# Autodesk Inventor assembly: FY 503 M
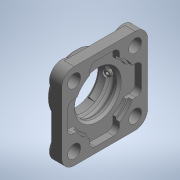
[picture p0: Inventor's stored thumbnail of the model, 180x180]
Saved by Autodesk Inventor 2020 (Build 240168000, 168)
## iProperties
Part Number: FY 503 M
Catalog Web Link: www.cadenas.de
Description: AFC_001-002_AFV_001-Square flanged housings for Y-bearings
Vendor: SKF
Document SubType Name: Assembly
Designer: partserver
Manufacturer: SKF
Mass: 280 g
Surface Area: 199.425 cm^2
Volume: 41.7862 cm^3
Density: 6.70078 g/cm^3
Category: PARTsolutions
Company: SKF
PSOL_IDENT_0: {$CADENAS_DATA\23d-libs\skf\bearings_units_and_housings\bearing_units\ball_bearing_units\y-housings\
PSOL_IDENT_1: afc_001-002_afv_001.prj},190 {VTYP=3D},{STYP=ASSTAB},{NB=FY 503 M},{LINA=FY 503 M},{NN=AFC_001-002_A
PSOL_IDENT_2: FV_001},{DATE=20.08.2020 13:45:12},{GEOMDATE=21.06.2019 12:06:37},{VERSION=},{LINEID=9370},{WBVAR=CO
PSOL_IDENT_3: VER},{WBNUMERIC=}  {NB=FY 503 M},{LINA=FY 503 M},{KT=DUMMY},{PRODUCTID=212600503},{DESIGNATION=FY 50
PSOL_IDENT_4: 3 M},{COVER=},{D=40.000},{DA=55.600},{DB1=50.000},{DB2=53.000},{DB=MIN},{A=26.000},{A1=11.000},{A2=1
PSOL_IDENT_5: 7.000},{A3=3.200},{A5=MIN},{J=54.000},{L=76.000},{N=11.500},{RG=1/4-28 UNF},{R1=19.000},{DN=6.500},{
PSOL_IDENT_6: SWN=7.000},{GN=1/4-28 SAE-LT},{J6=66.000},{J7=14.500},{N4=4.000},{MASS=0.280},{G=10.000},{GIN=0.375}
PSOL_IDENT_7: ,{HOUSING=},{EC=},{AEC=MIN},{DEC=MIN},{D1EC=MIN},{D2EC=MIN},{PPATH=square_flanged_housings_parts/afc
PSOL_IDENT_8: _001-002_afv_001_asmtpl.prj},{DESIGN=fy},{ECALG= '', 'No end cover'},{E=12},{TC=FY 503 M}
NB: FY 503 M
NN: AFC_001-002_AFV_001
NT: Square flanged housings for Y-bearings
NBSYN: $TC.
LINA: FY 503 M
CATALOG: SKF
DESIGNATION: FY 503 M
COVER: No end cover
D: 40
A: 26
L: 76
SUPPLIER: SKF
ARTICLENO: FY 503 M
BOMINFO: FY 503 M
CREATOR: CADENAS GmbH
Title: FY 503 M
Author: Cadenas PARTsolutions
Comments: Square flanged housings for Y-bearings
## Documents named in this file (3)
- C:\Users\Hesekiel\Desktop\Equatorial-Mount-MUM\Mechanika\Mechanizm elewacji Filip\CAD\FY 503 M\FY 503 M.iam
- C:\Users\Hesekiel\Desktop\Equatorial-Mount-MUM\Mechanika\Mechanizm elewacji Filip\CAD\FY 503 M\FY 503 M -Housing.ipt
- C:\Users\Hesekiel\Desktop\Equatorial-Mount-MUM\Mechanika\Mechanizm elewacji Filip\CAD\FY 503 M\1_4-28 SAE-LT.ipt
## Components (2 placed, 2 different names)
1. FY 503 M -Housing:1 — gn_XY@1 <-> gn_XY@2, gn_Z@1 <-> gn_Z@2, gn_YZ@1 <-> gn_YZ@2
2. 1_4-28 SAE-LT:1 — gn_XY@1 <-> gn_XY@2, gn_Z@1 <-> gn_Z@2, gn_YZ@1 <-> gn_YZ@2
## Relationships (3: Mate 2, Angle 1)
- gn_XY@1 <-> gn_XY@2 [Mate]: FY 503 M -Housing:1 ↔ 1_4-28 SAE-LT:1
- gn_Z@1 <-> gn_Z@2 [Mate]: FY 503 M -Housing:1 ↔ 1_4-28 SAE-LT:1
- gn_YZ@1 <-> gn_YZ@2 [Angle] (0 deg): FY 503 M -Housing:1 ↔ 1_4-28 SAE-LT:1
